# Autodesk Inventor assembly: A135
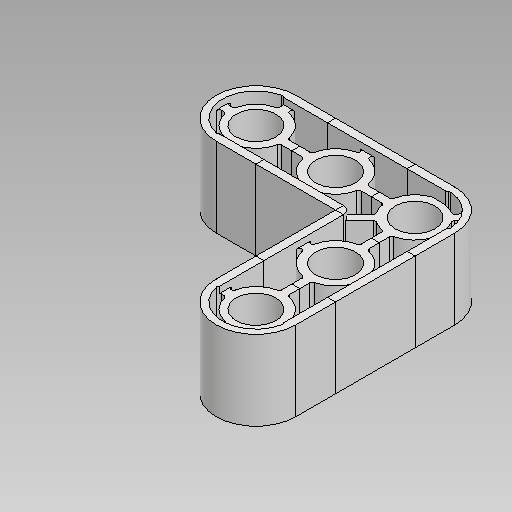
[picture p0: Inventor's stored thumbnail of the model, 512x512]
Saved by Autodesk Inventor 2020 (Build 240168000, 168)
## iProperties
Created: 2019-05-05
Part Number: A135
Document SubType Name: Assembly
Designer: Varga Daniel
Author: Varga Daniel
## Documents named in this file (5)
- C:\!_Dani\!_cloud\OneDrive\!_munka\Revolution\StructuralParts\Beams\Angled Beams\A90L.iam
- C:\!_Dani\!_cloud\OneDrive\!_munka\Revolution\StructuralParts\Beams\Beam_bent_base.ipt
- C:\!_Dani\!_cloud\OneDrive\!_munka\Revolution\StructuralParts\Beams\beam_single_end_part.ipt
- C:\!_Dani\!_cloud\OneDrive\!_munka\Revolution\StructuralParts\Beams\beam_single_inner_part.ipt
- C:\!_Dani\!_cloud\OneDrive\!_munka\Revolution\StructuralParts\Beams\Beam_bent_base\Beam_bent_base-90.ipt
## Components (5 placed, 3 different names)
1. Beam_bent_base-90:1 — Flush:12, Mate:4, Mate:5, Flush:13, Flush:14
2. beam_single_end_part:1 — Flush:1, Flush:2, Mate:1, Flush:13
3. beam_single_inner_part:2 — Flush:1, Flush:2, Mate:1, Flush:12, Mate:5
4. beam_single_end_part:2 — Flush:14
5. beam_single_inner_part:4 — Mate:4
## Relationships (11: Flush 7, Mate 4)
- Flush:1: beam_single_end_part:1 ↔ beam_single_inner_part:2
- Flush:2: beam_single_end_part:1 ↔ beam_single_inner_part:2
- Mate:1: beam_single_end_part:1 ↔ beam_single_inner_part:2
- [Flush]: beam_single_end_part:2 ↔ beam_single_inner_part:4
- [Flush]: beam_single_end_part:2 ↔ beam_single_inner_part:4
- [Mate]: beam_single_end_part:2 ↔ beam_single_inner_part:4
- Flush:12: Beam_bent_base-90:1 ↔ beam_single_inner_part:2
- Mate:4: Beam_bent_base-90:1 ↔ beam_single_inner_part:4
- Mate:5: Beam_bent_base-90:1 ↔ beam_single_inner_part:2
- Flush:13: Beam_bent_base-90:1 ↔ beam_single_end_part:1
- Flush:14: Beam_bent_base-90:1 ↔ beam_single_end_part:2
## Named parameters: d9_d0 = 0 mm, d10_d1 = 0 mm, d11_d2 = 0 mm
